# Autodesk Inventor assembly: SplayLeg
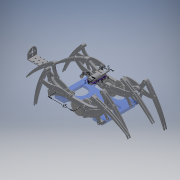
[picture p0: Inventor's stored thumbnail of the model, 180x180]
Saved by Autodesk Inventor 2017 (Build 210142000, 142)
## iProperties
Created: 2016-08-27
Part Number: SplayLeg
Document SubType Name: Assembly
Designer: Nic
Author: Nic
## Documents named in this file (12)
- C:\Users\Nic\Documents\TermiteBeest\SplayLeg.iam
- C:\Users\Nic\Documents\TermiteBeest\legFrame.ipt
- C:\Users\Nic\Documents\TermiteBeest\linkageC.ipt
- C:\Users\Nic\Documents\TermiteBeest\legB.ipt
- C:\Users\Nic\Documents\TermiteBeest\linkageB.ipt
- C:\Users\Nic\Documents\TermiteBeest\legA.ipt
- C:\Users\Nic\Documents\TermiteBeest\linkageA.ipt
- C:\Users\Nic\Documents\TermiteBeest\LegAssembly\Design Accelerator\Spur Gears1.iam
- C:\Users\Nic\Documents\TermiteBeest\baseplate.ipt
- C:\Users\Nic\Documents\TermiteBeest\Misc\MountingHub_3mm_M3.ipt
- C:\Users\Nic\Documents\TermiteBeest\Misc\MotorBracket_PL155D.ipt
- C:\Users\Nic\Documents\TermiteBeest\Misc\Motor_General.ipt
## Components (51 placed, 11 different names)
1. legFrame:1 — Rotational:4, Rotational:6, Rotational:8, Rotational:11, Rotational:12, Rotational:13, Rotational:18, Rotational:19, Rotational:20, Rotational:26, Rotational:27, Rotational:28, Rotational:33, Rotational:34, Insert:1, Insert:2
2. legB:1 — Rotational:3, Rotational:5, Rotational:9
3. linkageB:1 — Rotational:3, Rotational:4
4. legA:1 — Rotational:5, Rotational:7
5. linkageA:1 — Rotational:6, Rotational:7
6. linkageC:1 — Rotational:8, Rotational:9
7. linkageC:2 — Rotational:12, Rotational:14
8. linkageB:2 — Rotational:11, Rotational:15
9. linkageA:2 — Rotational:13, Rotational:16
10. legB:2 — Rotational:14, Rotational:15, Rotational:17
11. legA:2 — Rotational:16, Rotational:17
12. linkageC:3 — Rotational:18, Rotational:24
13. linkageA:3 — Rotational:19, Rotational:21
14. linkageB:3 — Rotational:20, Rotational:23
15. legA:3 — Rotational:21, Rotational:22
16. legB:3 — Rotational:22, Rotational:23, Rotational:24
17. linkageB:4 — Rotational:26, Rotational:31
18. linkageA:4 — Rotational:28, Rotational:29
19. linkageC:4 — Rotational:27, Rotational:30
20. legA:4 — Rotational:29, Rotational:32
21. legB:4 — Rotational:30, Rotational:31, Rotational:32
22. Spur Gears:1 [sub-assembly] — Rotational:33, Rotational:73
23. Spur Gears:2 [sub-assembly] — Rotational:34
24. baseplate:1 — Insert:1, Insert:2, Rotational:35, Rotational:59
25. linkageC:5 — Rotational:37, Rotational:48
26. linkageC:6 — Rotational:38, Rotational:52
27. legFrame:2 — Rotational:35, Rotational:37, Rotational:38, Rotational:39, Rotational:40, Rotational:44, Rotational:47, Rotational:55, Rotational:56, Rotational:58, Rotational:61, Rotational:62, Rotational:71
28. linkageA:6 — Rotational:39, Rotational:41
29. linkageA:7 — Rotational:40, Rotational:42
30. legA:5 — Rotational:42, Rotational:50
31. legA:6 — Rotational:41, Rotational:54
32. legB:5 — Rotational:48, Rotational:50, Rotational:51
33. legB:6 — Rotational:52, Rotational:53, Rotational:54
34. linkageB:5 — Rotational:44, Rotational:51
35. linkageB:6 — Rotational:47, Rotational:53
36. Spur Gears:3 [sub-assembly] — Rotational:55, Rotational:57, Rotational:72
37. Spur Gears:4 [sub-assembly] — Rotational:56
38. linkageC:7 — Rotational:58, Rotational:68
39. linkageC:8 — Rotational:57, Rotational:65
40. linkageB:7 — Rotational:59, Rotational:66
41. linkageB:8 — Rotational:69, Rotational:71
42. linkageA:8 — Rotational:61, Rotational:64
43. linkageA:9 — Rotational:62, Rotational:63
44. legA:7 — Rotational:64, Rotational:67
45. legA:8 — Rotational:63, Rotational:70
46. legB:7 — Rotational:65, Rotational:66, Rotational:67
47. legB:8 — Rotational:68, Rotational:69, Rotational:70
48. MountingHub_3mm_M3:1 — Rotational:72
49. MountingHub_3mm_M3:2 — Rotational:73
50. Motor_General:1
51. MotorBracket_PL155D:1
## Relationships (65: RevoluteJoint 63, Insert 2)
- Rotational:3 [RevoluteJoint]: legB:1 ↔ linkageB:1
- Rotational:4 [RevoluteJoint] (-1.5 mm): legFrame:1 ↔ linkageB:1
- Rotational:5 [RevoluteJoint]: legB:1 ↔ legA:1
- Rotational:6 [RevoluteJoint]: legFrame:1 ↔ linkageA:1
- Rotational:7 [RevoluteJoint]: legA:1 ↔ linkageA:1
- Rotational:8 [RevoluteJoint]: legFrame:1 ↔ linkageC:1
- Rotational:9 [RevoluteJoint] (-1.5 mm): legB:1 ↔ linkageC:1
- Rotational:11 [RevoluteJoint] (-1.5 mm): legFrame:1 ↔ linkageB:2
- Rotational:12 [RevoluteJoint]: legFrame:1 ↔ linkageC:2
- Rotational:13 [RevoluteJoint]: legFrame:1 ↔ linkageA:2
- Rotational:14 [RevoluteJoint] (-1.5 mm): linkageC:2 ↔ legB:2
- Rotational:15 [RevoluteJoint]: linkageB:2 ↔ legB:2
- Rotational:16 [RevoluteJoint]: linkageA:2 ↔ legA:2
- Rotational:17 [RevoluteJoint]: legB:2 ↔ legA:2
- Rotational:18 [RevoluteJoint] (-7 mm): legFrame:1 ↔ linkageC:3
- Rotational:19 [RevoluteJoint] (-7 mm): legFrame:1 ↔ linkageA:3
- Rotational:20 [RevoluteJoint] (-8.5 mm): legFrame:1 ↔ linkageB:3
- Rotational:21 [RevoluteJoint]: linkageA:3 ↔ legA:3
- Rotational:22 [RevoluteJoint]: legA:3 ↔ legB:3
- Rotational:23 [RevoluteJoint]: linkageB:3 ↔ legB:3
- Rotational:24 [RevoluteJoint] (-1.5 mm): linkageC:3 ↔ legB:3
- Rotational:26 [RevoluteJoint] (-8.5 mm): legFrame:1 ↔ linkageB:4
- Rotational:27 [RevoluteJoint] (-7 mm): legFrame:1 ↔ linkageC:4
- Rotational:28 [RevoluteJoint] (-7 mm): legFrame:1 ↔ linkageA:4
- Rotational:29 [RevoluteJoint]: linkageA:4 ↔ legA:4
- Rotational:30 [RevoluteJoint] (-1.5 mm): linkageC:4 ↔ legB:4
- Rotational:31 [RevoluteJoint]: linkageB:4 ↔ legB:4
- Rotational:32 [RevoluteJoint]: legA:4 ↔ legB:4
- Rotational:33 [RevoluteJoint]: legFrame:1 ↔ Spur Gears:1
- Rotational:34 [RevoluteJoint]: legFrame:1 ↔ Spur Gears:2
- Insert:1: legFrame:1 ↔ baseplate:1
- Insert:2: legFrame:1 ↔ baseplate:1
- Rotational:35 [RevoluteJoint]: baseplate:1 ↔ legFrame:2
- Rotational:37 [RevoluteJoint]: linkageC:5 ↔ legFrame:2
- Rotational:38 [RevoluteJoint]: linkageC:6 ↔ legFrame:2
- Rotational:39 [RevoluteJoint]: legFrame:2 ↔ linkageA:6
- Rotational:40 [RevoluteJoint]: legFrame:2 ↔ linkageA:7
- Rotational:41 [RevoluteJoint]: linkageA:6 ↔ legA:6
- Rotational:42 [RevoluteJoint]: linkageA:7 ↔ legA:5
- Rotational:44 [RevoluteJoint] (-1.5 mm): legFrame:2 ↔ linkageB:5
- Rotational:47 [RevoluteJoint] (-1.5 mm): legFrame:2 ↔ linkageB:6
- Rotational:48 [RevoluteJoint] (-1.5 mm): linkageC:5 ↔ legB:5
- Rotational:50 [RevoluteJoint]: legA:5 ↔ legB:5
- Rotational:51 [RevoluteJoint]: legB:5 ↔ linkageB:5
- Rotational:52 [RevoluteJoint] (-1.5 mm): linkageC:6 ↔ legB:6
- Rotational:53 [RevoluteJoint]: legB:6 ↔ linkageB:6
- Rotational:54 [RevoluteJoint]: legA:6 ↔ legB:6
- Rotational:55 [RevoluteJoint]: legFrame:2 ↔ Spur Gears:3
- Rotational:56 [RevoluteJoint]: legFrame:2 ↔ Spur Gears:4
- Rotational:57 [RevoluteJoint] (-5.5 mm): Spur Gears:3 ↔ linkageC:8
- Rotational:58 [RevoluteJoint] (-7 mm): legFrame:2 ↔ linkageC:7
- Rotational:59 [RevoluteJoint] (-5.5 mm): baseplate:1 ↔ linkageB:7
- Rotational:61 [RevoluteJoint] (-7 mm): legFrame:2 ↔ linkageA:8
- Rotational:62 [RevoluteJoint] (-7 mm): legFrame:2 ↔ linkageA:9
- Rotational:63 [RevoluteJoint]: linkageA:9 ↔ legA:8
- Rotational:64 [RevoluteJoint]: linkageA:8 ↔ legA:7
- Rotational:65 [RevoluteJoint] (-1.5 mm): linkageC:8 ↔ legB:7
- Rotational:66 [RevoluteJoint]: linkageB:7 ↔ legB:7
- Rotational:67 [RevoluteJoint]: legA:7 ↔ legB:7
- Rotational:68 [RevoluteJoint] (-1.5 mm): linkageC:7 ↔ legB:8
- Rotational:69 [RevoluteJoint]: linkageB:8 ↔ legB:8
- Rotational:70 [RevoluteJoint]: legA:8 ↔ legB:8
- Rotational:71 [RevoluteJoint] (-8.5 mm): legFrame:2 ↔ linkageB:8
- Rotational:72 [RevoluteJoint]: Spur Gears:3 ↔ MountingHub_3mm_M3:1
- Rotational:73 [RevoluteJoint]: Spur Gears:1 ↔ MountingHub_3mm_M3:2
